# Autodesk Inventor assembly: YAxis_Carriage
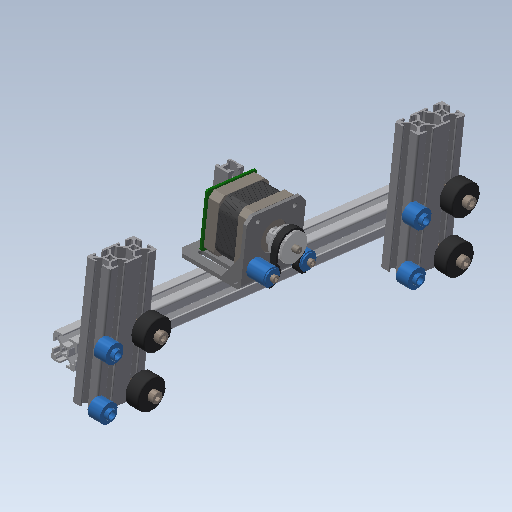
[picture p0: Inventor's stored thumbnail of the model, 512x512]
Saved by Autodesk Inventor 2021 (Build 250183000, 183)
## iProperties
Created: 2021-02-02
Part Number: YAxis_Carriage
Document SubType Name: Assembly
Designer: Jorian Brusind
Author: Jorian Brusind
## Documents named in this file (12)
- C:\Users\Jorian Brusind\Documents\GitHub\PersonalProjects\HyperRail\Inventor Files\YAxis_Carriage.iam
- C:\Users\Jorian Brusind\Documents\GitHub\PersonalProjects\Inventor Projects\Useful models\8020_Sets\IPT_20_Series\IPT_20_Series\20-2020_300mm.ipt
- C:\Users\Jorian Brusind\Documents\GitHub\PersonalProjects\Inventor Projects\Useful models\NEMA_Steppers\nema-17-stepper-motor-with-v2-damper-1.snapshot.3\Nema 17  Stepper Motor length 34mm.ipt
- C:\Users\Jorian Brusind\Documents\GitHub\PersonalProjects\Inventor Projects\Useful models\NEMA_Steppers\nema-17-steel-motor-mount-1.snapshot.2\NEMA17 - Steel Motor Mount.ipt
- C:\Users\Jorian Brusind\Documents\GitHub\PersonalProjects\HyperRail\Inventor Files\SmallBelt_Pulley.ipt
- C:\Users\Jorian Brusind\Documents\GitHub\PersonalProjects\HyperRail\Inventor Files\Idle_pulley_small.ipt
- C:\Users\Jorian Brusind\Documents\GitHub\PersonalProjects\Inventor Projects\Useful models\683ZZBallBearing.ipt
- C:\Users\Jorian Brusind\Documents\GitHub\PersonalProjects\HyperRail\Inventor Files\3mmSpacer.ipt
- C:\Users\Jorian Brusind\Documents\GitHub\PersonalProjects\Inventor Projects\Useful models\Metric bolt\Bolt M3 30mm.ipt
- C:\Users\Jorian Brusind\Documents\GitHub\PersonalProjects\HyperRail\Inventor Files\small_belt_loop.ipt
- C:\Users\Jorian Brusind\Documents\GitHub\PersonalProjects\HyperRail\Inventor Files\Roller_Bracket_20mm.iam
- C:\Users\Jorian Brusind\Documents\GitHub\PersonalProjects\HyperRail\PCB Files\Integrated Stepper Motor Driver\ExportSTEP\Main.iam
## Components (18 placed, 11 different names)
1. 20-2020_300mm:1 — Mate:3, Flush:8, Mate:41, Flush:9, Flush:12
2. Nema 17  Stepper Motor length 34mm:1 — Mate:4, Mate:5, Mate:6, Mate:13, Mate:14, Mate:36, Mate:42, Flush:14, Flush:15
3. NEMA17 - Steel Motor Mount:1 — Mate:3, Mate:4, Mate:5, Mate:6, Mate:20, Mate:21, Mate:23, Mate:35
4. SmallBelt_Pulley:1 — Mate:13, Mate:14, Mate:37, Flush:13
5. Idle_pulley_small:1 — Mate:18, Flush:6, Mate:24
6. Idle_pulley_small:2 — Mate:19, Flush:7, Mate:30
7. 683ZZBallBearing:1 — Mate:18, Flush:6, Mate:27, Mate:29
8. 683ZZBallBearing:2 — Mate:19, Flush:7, Mate:31, Mate:33
9. 3mmSpacer:1 — Mate:32, Mate:33, Mate:35
10. 3mmSpacer:2 — Mate:22, Mate:23, Mate:27
11. 3mmSpacer:3 — Mate:30, Mate:31, Mate:32, Mate:34, Mate:40
12. 3mmSpacer:4 — Mate:26, Mate:28, Mate:29, Mate:39
13. Bolt M3 30mm:1 — Mate:20, Mate:22, Mate:24, Mate:26, Mate:28, Mate:39
14. Bolt M3 30mm:2 — Mate:21, Mate:34, Mate:38, Mate:40
15. small_belt_loop:1 — Mate:36, Mate:37, Mate:38
16. Roller_Bracket_20mm:1 [sub-assembly] — Flush:10, Flush:11, Flush:12, Flush:13
17. Roller_Bracket_20mm:2 [sub-assembly] — Flush:8, Mate:41, Flush:9, Flush:10, Flush:11
18. Main:1 [sub-assembly] — Mate:42, Flush:14, Flush:15
## Relationships (40: Mate 30, Flush 10)
- Mate:3 (3 mm): 20-2020_300mm:1 ↔ NEMA17 - Steel Motor Mount:1
- Mate:4: Nema 17  Stepper Motor length 34mm:1 ↔ NEMA17 - Steel Motor Mount:1
- Mate:5: Nema 17  Stepper Motor length 34mm:1 ↔ NEMA17 - Steel Motor Mount:1
- Mate:6: Nema 17  Stepper Motor length 34mm:1 ↔ NEMA17 - Steel Motor Mount:1
- Mate:13: Nema 17  Stepper Motor length 34mm:1 ↔ SmallBelt_Pulley:1
- Mate:14: Nema 17  Stepper Motor length 34mm:1 ↔ SmallBelt_Pulley:1
- Mate:18: Idle_pulley_small:1 ↔ 683ZZBallBearing:1
- Flush:6 (5 mm): Idle_pulley_small:1 ↔ 683ZZBallBearing:1
- Mate:19: Idle_pulley_small:2 ↔ 683ZZBallBearing:2
- Flush:7 (5 mm): Idle_pulley_small:2 ↔ 683ZZBallBearing:2
- Mate:20: NEMA17 - Steel Motor Mount:1 ↔ Bolt M3 30mm:1
- Mate:21: NEMA17 - Steel Motor Mount:1 ↔ Bolt M3 30mm:2
- Mate:22: 3mmSpacer:2 ↔ Bolt M3 30mm:1
- Mate:23: NEMA17 - Steel Motor Mount:1 ↔ 3mmSpacer:2
- Mate:24: Idle_pulley_small:1 ↔ Bolt M3 30mm:1
- Mate:26: 3mmSpacer:4 ↔ Bolt M3 30mm:1
- Mate:27: 683ZZBallBearing:1 ↔ 3mmSpacer:2
- Mate:28: 3mmSpacer:4 ↔ Bolt M3 30mm:1
- Mate:29: 683ZZBallBearing:1 ↔ 3mmSpacer:4
- Mate:30: Idle_pulley_small:2 ↔ 3mmSpacer:3
- Mate:31: 683ZZBallBearing:2 ↔ 3mmSpacer:3
- Mate:32: 3mmSpacer:1 ↔ 3mmSpacer:3
- Mate:33: 683ZZBallBearing:2 ↔ 3mmSpacer:1
- Mate:34: 3mmSpacer:3 ↔ Bolt M3 30mm:2
- Mate:35: NEMA17 - Steel Motor Mount:1 ↔ 3mmSpacer:1
- Mate:36: Nema 17  Stepper Motor length 34mm:1 ↔ small_belt_loop:1
- Mate:37 (2 mm): SmallBelt_Pulley:1 ↔ small_belt_loop:1
- Mate:38: Bolt M3 30mm:2 ↔ small_belt_loop:1
- Mate:39: 3mmSpacer:4 ↔ Bolt M3 30mm:1
- Mate:40: 3mmSpacer:3 ↔ Bolt M3 30mm:2
- Flush:8 (-20 mm): 20-2020_300mm:1 ↔ Roller_Bracket_20mm:2
- Mate:41: 20-2020_300mm:1 ↔ Roller_Bracket_20mm:2
- Flush:9: 20-2020_300mm:1 ↔ Roller_Bracket_20mm:2
- Flush:10: Roller_Bracket_20mm:1 ↔ Roller_Bracket_20mm:2
- Flush:11: Roller_Bracket_20mm:1 ↔ Roller_Bracket_20mm:2
- Flush:12: 20-2020_300mm:1 ↔ Roller_Bracket_20mm:1
- Flush:13: SmallBelt_Pulley:1 ↔ Roller_Bracket_20mm:1
- Mate:42: Nema 17  Stepper Motor length 34mm:1 ↔ Main:1
- Flush:14: Nema 17  Stepper Motor length 34mm:1 ↔ Main:1
- Flush:15: Nema 17  Stepper Motor length 34mm:1 ↔ Main:1
